# Autodesk Inventor assembly: cam_set
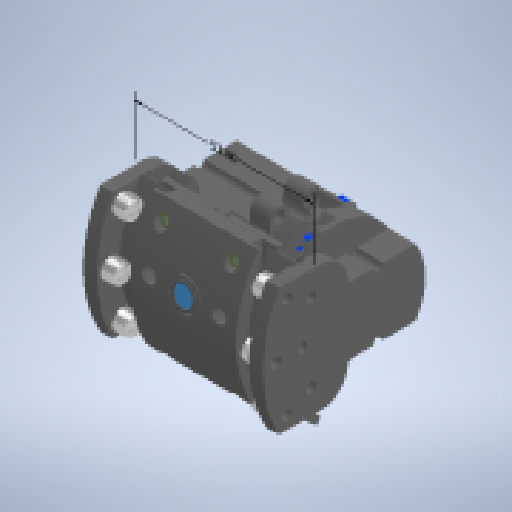
[picture p0: Inventor's stored thumbnail of the model, 512x512]
Saved by Autodesk Inventor 2024.1 (Build 281209000, 209)
## iProperties
Created: 2025-01-10
Part Number: cam_set
Document SubType Name: Assembly
Designer: hibik
Author: hibik
## Documents named in this file (7)
- C:\Users\hibik\Documents\Robomech\RESCUE\ORCA\hard\camera\cam_set.iam
- C:\Users\hibik\Documents\Robomech\RESCUE\ORCA\hard\camera\cam_set_cover_right.ipt
- C:\Users\hibik\Documents\Robomech\RESCUE\ORCA\hard\std_parts\sg90_Tower_Pro.ipt
- C:\Users\hibik\Documents\Robomech\RESCUE\ORCA\hard\camera\geard_hone.ipt
- C:\Users\hibik\Documents\Robomech\RESCUE\ORCA\hard\std_parts\bearing_3_6_2.5.ipt
- C:\Users\hibik\Documents\Robomech\RESCUE\ORCA\hard\camera\cam_set_cover_left.ipt
- C:\Users\hibik\Documents\Robomech\RESCUE\ORCA\hard\camera\cam.iam
## Components (17 placed, 6 different names)
1. cam_set_cover_right:1 — メイト:1, フラッシュ:1, フラッシュ:2, メイト:2, メイト:3, メイト:4, フラッシュ:3, メイト:5, 正接:1, フラッシュ:4, 挿入:9, 挿入:16, 挿入:17, 挿入:18, 挿入:19, 挿入:20, 挿入:21
2. sg90_Tower_Pro:1 — メイト:2, メイト:3, メイト:4, 挿入:1, フラッシュ:3
3. geard_hone:1 — 挿入:1
4. bearing_3_6_2.5:1 — 挿入:19
5. bearing_3_6_2.5:2 — 挿入:21
6. bearing_3_6_2.5:3 — 挿入:18
7. bearing_3_6_2.5:4 — 挿入:16
8. bearing_3_6_2.5:5 — 挿入:17
9. bearing_3_6_2.5:6 — 挿入:20
10. cam_set_cover_left:1 — メイト:5, 正接:1, フラッシュ:4, 挿入:10, 挿入:11, 挿入:12, 挿入:13, 挿入:14, 挿入:15
11. cam:1 [sub-assembly] — 挿入:9
12. bearing_3_6_2.5:7 — 挿入:11
13. bearing_3_6_2.5:8 — 挿入:10
14. bearing_3_6_2.5:9 — 挿入:12
15. bearing_3_6_2.5:10 — 挿入:13
16. bearing_3_6_2.5:11 — 挿入:15
17. bearing_3_6_2.5:12 — 挿入:14
## Relationships (24: Insert 14, Mate 5, Flush 4, Tangent 1)
- メイト:1 [Mate] (22.9 mm): cam_set_cover_right:1
- フラッシュ:1 [Flush]: cam_set_cover_right:1
- フラッシュ:2 [Flush]: cam_set_cover_right:1
- メイト:2 [Mate]: cam_set_cover_right:1 ↔ sg90_Tower_Pro:1
- メイト:3 [Mate] (0.1 mm): cam_set_cover_right:1 ↔ sg90_Tower_Pro:1
- メイト:4 [Mate] (0.1 mm): cam_set_cover_right:1 ↔ sg90_Tower_Pro:1
- 挿入:1 [Insert]: sg90_Tower_Pro:1 ↔ geard_hone:1
- フラッシュ:3 [Flush]: cam_set_cover_right:1 ↔ sg90_Tower_Pro:1
- メイト:5 [Mate] (45.8 mm): cam_set_cover_right:1 ↔ cam_set_cover_left:1
- 正接:1 [Tangent]: cam_set_cover_right:1 ↔ cam_set_cover_left:1
- フラッシュ:4 [Flush]: cam_set_cover_right:1 ↔ cam_set_cover_left:1
- 挿入:9 [Insert]: cam_set_cover_right:1 ↔ cam:1
- 挿入:10 [Insert]: cam_set_cover_left:1 ↔ bearing_3_6_2.5:8
- 挿入:11 [Insert]: cam_set_cover_left:1 ↔ bearing_3_6_2.5:7
- 挿入:12 [Insert]: cam_set_cover_left:1 ↔ bearing_3_6_2.5:9
- 挿入:13 [Insert]: cam_set_cover_left:1 ↔ bearing_3_6_2.5:10
- 挿入:14 [Insert]: cam_set_cover_left:1 ↔ bearing_3_6_2.5:12
- 挿入:15 [Insert]: cam_set_cover_left:1 ↔ bearing_3_6_2.5:11
- 挿入:16 [Insert]: cam_set_cover_right:1 ↔ bearing_3_6_2.5:4
- 挿入:17 [Insert]: cam_set_cover_right:1 ↔ bearing_3_6_2.5:5
- 挿入:18 [Insert]: cam_set_cover_right:1 ↔ bearing_3_6_2.5:3
- 挿入:19 [Insert]: cam_set_cover_right:1 ↔ bearing_3_6_2.5:1
- 挿入:20 [Insert]: cam_set_cover_right:1 ↔ bearing_3_6_2.5:6
- 挿入:21 [Insert]: cam_set_cover_right:1 ↔ bearing_3_6_2.5:2
